# Autodesk Inventor assembly: DHT11-Exploded View
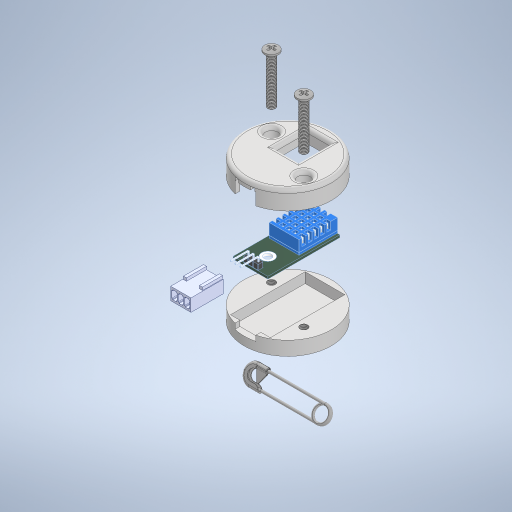
[picture p0: Inventor's stored thumbnail of the model, 512x512]
Saved by Autodesk Inventor 2023 (Build 270158000, 158)
## iProperties
Created: 2024-03-19
Part Number: DHT11-Exploded View
Document SubType Name: Assembly
Designer: ongyu
Author: ongyu
## Documents named in this file (7)
- C:\Users\ongyu\OneDrive\Documents\Inventor\FYP\DHT11-Shell\DHT11-Exploded-View.iam
- C:\Users\ongyu\OneDrive\Documents\Inventor\FYP\DHT11-Shell\01 - DHT11-Case-Btm.ipt
- C:\Users\ongyu\OneDrive\Documents\Inventor\FYP\DHT11-Shell\02 - DHT11-Case-Top.ipt
- C:\Users\ongyu\OneDrive\Documents\Inventor\FYP\DHT11-Shell\03 - DHT11.ipt
- C:\Users\ongyu\OneDrive\Documents\Inventor\FYP\DHT11-Shell\04 - M3-8mm.ipt
- C:\Users\ongyu\OneDrive\Documents\Inventor\FYP\DHT11-Shell\05 - Three-Pin-Connector.ipt
- C:\Users\ongyu\OneDrive\Documents\Inventor\FYP\DHT11-Shell\06 - Safety-Pin.ipt
## Components (7 placed, 6 different names)
1. 01 - DHT11-Case-Btm:1 — Flush:1, Flush:2, Flush:3, Insert:1, Flush:4, Mate:1, Mate:4
2. 02 - DHT11-Case-Top:1 — Insert:1, Insert:2, Insert:3
3. 03 - DHT11:1 — Flush:4, Mate:1, Flush:5, Mate:3
4. 04 - M3-8mm:1 — Insert:2
5. 05 - Three-Pin-Connector:1 — Mate:2, Mate:3
6. 04 - M3-8mm:2 — Insert:3
7. 06 - Safety-Pin:1 — Mate:4, Flush:6
## Relationships (13: Flush 6, Mate 4, Insert 3)
- Flush:1: 01 - DHT11-Case-Btm:1
- Flush:2: 01 - DHT11-Case-Btm:1
- Flush:3: 01 - DHT11-Case-Btm:1
- Insert:1 (45 mm): 01 - DHT11-Case-Btm:1 ↔ 02 - DHT11-Case-Top:1
- Flush:4 (-25 mm): 01 - DHT11-Case-Btm:1 ↔ 03 - DHT11:1
- Mate:1: 01 - DHT11-Case-Btm:1 ↔ 03 - DHT11:1
- Flush:5: 03 - DHT11:1
- Mate:2: 05 - Three-Pin-Connector:1
- Mate:3: 03 - DHT11:1 ↔ 05 - Three-Pin-Connector:1
- Insert:2 (-10 mm): 02 - DHT11-Case-Top:1 ↔ 04 - M3-8mm:1
- Insert:3 (10 mm): 02 - DHT11-Case-Top:1 ↔ 04 - M3-8mm:2
- Mate:4 (25 mm): 01 - DHT11-Case-Btm:1 ↔ 06 - Safety-Pin:1
- Flush:6: 06 - Safety-Pin:1
